# Autodesk Inventor assembly: EsagonoScreeenChiuso
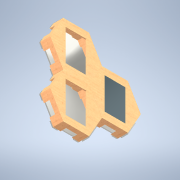
[picture p0: Inventor's stored thumbnail of the model, 180x180]
Saved by Autodesk Inventor 2020 (Build 240168000, 168)
## iProperties
Created: 2020-04-22
Part Number: EsagonoScreeenChiuso
Document SubType Name: Assembly
Designer: Samuele
Author: Samuele
## Documents named in this file (4)
- C:\EsagoniMalsani\ModelliComponenti\EsagonoScreeenChiuso.iam
- C:\EsagoniMalsani\ModelliComponenti\HexagoneBack.ipt
- C:\EsagoniMalsani\ModelliComponenti\Hexagone.ipt
- C:\EsagoniMalsani\ModelliComponenti\TouchLCD.ipt
## Components (7 placed, 3 different names)
1. HexagoneBack:1 — Flush:1, Flush:2, Mate:1
2. Hexagone:1 — Flush:1, Flush:2, Mate:1, Mate:4, Flush:7, Mate:5, Mate:7
3. HexagoneBack:5
4. Hexagone:5 — Flush:8, Mate:6, Mate:7, Flush:9, Mate:8, Mate:9
5. HexagoneBack:6 — Mate:5
6. Hexagone:6 — Mate:4, Flush:7, Flush:8, Mate:6
7. TouchLCD:1 — Flush:9, Mate:8, Mate:9
## Relationships (18: Flush 9, Mate 9)
- Flush:1: HexagoneBack:1 ↔ Hexagone:1
- Flush:2: HexagoneBack:1 ↔ Hexagone:1
- Mate:1: HexagoneBack:1 ↔ Hexagone:1
- [Flush]: HexagoneBack:5 ↔ Hexagone:5
- [Flush]: HexagoneBack:5 ↔ Hexagone:5
- [Mate]: HexagoneBack:5 ↔ Hexagone:5
- [Flush]: HexagoneBack:6 ↔ Hexagone:6
- [Flush]: HexagoneBack:6 ↔ Hexagone:6
- [Mate]: HexagoneBack:6 ↔ Hexagone:6
- Mate:4: Hexagone:1 ↔ Hexagone:6
- Flush:7: Hexagone:1 ↔ Hexagone:6
- Mate:5: Hexagone:1 ↔ HexagoneBack:6
- Flush:8: Hexagone:5 ↔ Hexagone:6
- Mate:6: Hexagone:5 ↔ Hexagone:6
- Mate:7: Hexagone:1 ↔ Hexagone:5
- Flush:9: Hexagone:5 ↔ TouchLCD:1
- Mate:8: Hexagone:5 ↔ TouchLCD:1
- Mate:9: Hexagone:5 ↔ TouchLCD:1
## Named parameters: d3_d2 = 0 mm, d4_d0 = 0 mm, d5_d1 = 0 mm, d6_d2 = 0 mm, d7_d0 = 0 mm, d8_d1 = 0 mm
